# Autodesk Inventor assembly: Hopper Linear Guide
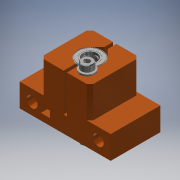
[picture p0: Inventor's stored thumbnail of the model, 180x180]
Saved by Autodesk Inventor 2018 (Build 220112000, 112)
## iProperties
Created: 2017-09-26
Part Number: Hopper Linear Guide
Document SubType Name: Assembly
Designer: Gabriel Smolnycki
Author: Gabriel Smolnycki
## Documents named in this file (6)
- H:\dev\planb\mechanics\V1INV\Subassemblies\Hopper Linear Guide.iam
- H:\dev\planb\mechanics\V1INV\Hopper\Hopper Linear Bearing Holder.ipt
- H:\dev\planb\mechanics\V1INV\Hardware\8x25 Linear Bearing (63255K45).ipt
- H:\dev\planb\mechanics\V1INV\Hardware\M4x40 SS SHCS.ipt
- H:\dev\planb\mechanics\V1INV\Hardware\M4 SS Washer.ipt
- H:\dev\planb\mechanics\V1INV\Hardware\M4 SS Nut.ipt
## Components (6 placed, 5 different names)
1. Hopper Linear Bearing Holder:1 — Mate:1, Insert:1, Insert:3, Insert:17
2. 8x25 Linear Bearing (63255K45):1 — Mate:1, Insert:1
3. M4x40 SS SHCS:1 — Insert:18
4. M4 SS Washer:1 — Insert:3, Insert:4
5. M4 SS Washer:2 — Insert:17, Insert:18
6. M4 SS Nut:1 — Insert:4
## Relationships (6: Insert 5, Mate 1)
- Mate:1: Hopper Linear Bearing Holder:1 ↔ 8x25 Linear Bearing (63255K45):1
- Insert:1: Hopper Linear Bearing Holder:1 ↔ 8x25 Linear Bearing (63255K45):1
- Insert:3: Hopper Linear Bearing Holder:1 ↔ M4 SS Washer:1
- Insert:4: M4 SS Washer:1 ↔ M4 SS Nut:1
- Insert:17: Hopper Linear Bearing Holder:1 ↔ M4 SS Washer:2
- Insert:18: M4x40 SS SHCS:1 ↔ M4 SS Washer:2
